# Autodesk Inventor assembly: WearableAssembly
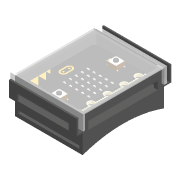
[picture p0: Inventor's stored thumbnail of the model, 180x180]
Saved by Autodesk Inventor 2022 (Build 260153000, 153)
## iProperties
Created: 2021-06-28
Part Number: WearableAssembly
Document SubType Name: Assembly
Designer: Prajwal Patil
Author: Prajwal Patil
## Documents named in this file (4)
- C:\Users\Prajwal Patil\Desktop\Wearable\WearableAssembly.iam
- C:\Users\Prajwal Patil\Desktop\Wearable\wear1.ipt
- C:\Users\Prajwal Patil\Desktop\Wearable\Microbit\BBC microbit V1.5.iam
- C:\Users\Prajwal Patil\Desktop\Wearable\glasscover_MIR1.ipt
## Components (3 placed, 3 different names)
1. wear1:1 — Mate:4, Mate:5, Mate:6
2. BBC microbit V1.5:1 [sub-assembly] — Mate:5, Mate:6
3. glasscover_MIR1:1 — Mate:4
## Relationships (3: Mate 3)
- Mate:4: wear1:1 ↔ glasscover_MIR1:1
- Mate:5: wear1:1 ↔ BBC microbit V1.5:1
- Mate:6: wear1:1 ↔ BBC microbit V1.5:1
